# Autodesk Inventor assembly: FlyWheelAssembly3_Jan23
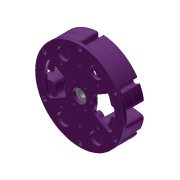
[picture p0: Inventor's stored thumbnail of the model, 180x180]
Saved by Autodesk Inventor 2012 (Build 160160000, 160)
## iProperties
Created: 2012-01-24
Part Number: FlyWheelAssembly3_Jan23
Document SubType Name: Assembly
Designer: JesseK
Mass: 737.914 g
Surface Area: 780.199 cm^2
Volume: 272.293 cm^3
Density: 2.71 g/cm^3
Author: JesseK
## Documents named in this file (4)
- Z:\UserData\Documents\Inventor\team1885frc\Robot2012\Shooter\FlyWheelAssembly3_Jan23.iam
- Z:\UserData\Documents\Inventor\team1885frc\Robot2012\Shooter\FlyWheel_Base_Jan21.ipt
- Z:\UserData\Documents\Inventor\team1885frc\Robot2012\Shooter\IFI_Wheel_Weight_8in.ipt
- Z:\UserData\Documents\Inventor\team1885frc\AndyMark\500EX-Key-Hub.ipt
## Components (6 placed, 3 different names)
1. FlyWheel_Base_Jan21:1 — Mate:1, Mate:2, Mate:3, Mate:6, Mate:7, Mate:8, Mate:9, Mate:10, Mate:11, Mate:14, Mate:15
2. IFI_Wheel_Weight_8in:1 — Mate:1, Mate:2, Mate:12
3. IFI_Wheel_Weight_8in:2 — Mate:3, Mate:10, Mate:11, Mate:13
4. IFI_Wheel_Weight_8in:3 — Mate:6, Mate:7, Mate:13
5. IFI_Wheel_Weight_8in:4 — Mate:8, Mate:9, Mate:12
6. 500EX-Key-Hub:1 — Mate:14, Mate:15
## Relationships (13: Mate 13)
- Mate:1: FlyWheel_Base_Jan21:1 ↔ IFI_Wheel_Weight_8in:1
- Mate:2: FlyWheel_Base_Jan21:1 ↔ IFI_Wheel_Weight_8in:1
- Mate:3: FlyWheel_Base_Jan21:1 ↔ IFI_Wheel_Weight_8in:2
- Mate:6: FlyWheel_Base_Jan21:1 ↔ IFI_Wheel_Weight_8in:3
- Mate:7: FlyWheel_Base_Jan21:1 ↔ IFI_Wheel_Weight_8in:3
- Mate:8: FlyWheel_Base_Jan21:1 ↔ IFI_Wheel_Weight_8in:4
- Mate:9: FlyWheel_Base_Jan21:1 ↔ IFI_Wheel_Weight_8in:4
- Mate:10: FlyWheel_Base_Jan21:1 ↔ IFI_Wheel_Weight_8in:2
- Mate:11: FlyWheel_Base_Jan21:1 ↔ IFI_Wheel_Weight_8in:2
- Mate:12: IFI_Wheel_Weight_8in:1 ↔ IFI_Wheel_Weight_8in:4
- Mate:13: IFI_Wheel_Weight_8in:2 ↔ IFI_Wheel_Weight_8in:3
- Mate:14: FlyWheel_Base_Jan21:1 ↔ 500EX-Key-Hub:1
- Mate:15: FlyWheel_Base_Jan21:1 ↔ 500EX-Key-Hub:1
